# Autodesk Inventor assembly: outer
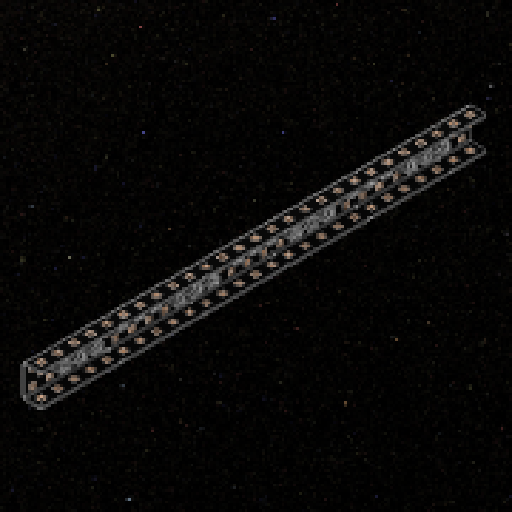
[picture p0: Inventor's stored thumbnail of the model, 512x512]
Saved by Autodesk Inventor 2024 (Build 280153000, 153)
## iProperties
Created: 2024-02-24
Part Number: outer
Document SubType Name: Assembly
Designer: Averey Ku
Author: Averey Ku
## Documents named in this file (3)
- D:\vex_robotics\hardware\cad\lil_zoom\chassis\drivebay\outer.iam
- D:\vex_robotics\hardware\cad\VEX-CAD-Inventor-1.41\Structure\C Channel\Aluminum 1x2x1\Alu C 1x2x1x27.ipt
- D:\vex_robotics\hardware\cad\VEX-CAD-Inventor-1.41\Motion\Shaft LS\Bearing Flat Low Profile.ipt
## Components (8 placed, 2 different names)
1. Alu C 1x2x1x27:1 — Insert:1, Mate:1, Insert:2, Mate:2, Insert:3, Mate:3, Insert:4, Mate:4, Insert:5, Mate:5, Insert:6, Mate:6, Insert:7, Mate:7
2. Bearing Flat Low Profile:1 — Insert:1, Mate:1
3. Bearing Flat Low Profile:2 — Insert:3, Mate:3
4. Bearing Flat Low Profile:3 — Insert:2, Mate:2
5. Bearing Flat Low Profile:4 — Insert:5, Mate:5
6. Bearing Flat Low Profile:5 — Insert:6, Mate:6
7. Bearing Flat Low Profile:6 — Insert:7, Mate:7
8. Bearing Flat Low Profile:7 — Insert:4, Mate:4
## Relationships (14: Insert 7, Mate 7)
- Insert:1: Alu C 1x2x1x27:1 ↔ Bearing Flat Low Profile:1
- Mate:1: Alu C 1x2x1x27:1 ↔ Bearing Flat Low Profile:1
- Insert:2: Alu C 1x2x1x27:1 ↔ Bearing Flat Low Profile:3
- Mate:2: Alu C 1x2x1x27:1 ↔ Bearing Flat Low Profile:3
- Insert:3: Alu C 1x2x1x27:1 ↔ Bearing Flat Low Profile:2
- Mate:3: Alu C 1x2x1x27:1 ↔ Bearing Flat Low Profile:2
- Insert:4: Alu C 1x2x1x27:1 ↔ Bearing Flat Low Profile:7
- Mate:4: Alu C 1x2x1x27:1 ↔ Bearing Flat Low Profile:7
- Insert:5: Alu C 1x2x1x27:1 ↔ Bearing Flat Low Profile:4
- Mate:5: Alu C 1x2x1x27:1 ↔ Bearing Flat Low Profile:4
- Insert:6: Alu C 1x2x1x27:1 ↔ Bearing Flat Low Profile:5
- Mate:6: Alu C 1x2x1x27:1 ↔ Bearing Flat Low Profile:5
- Insert:7: Alu C 1x2x1x27:1 ↔ Bearing Flat Low Profile:6
- Mate:7: Alu C 1x2x1x27:1 ↔ Bearing Flat Low Profile:6
